# Autodesk Inventor assembly: Pata - Ensamble Trasero
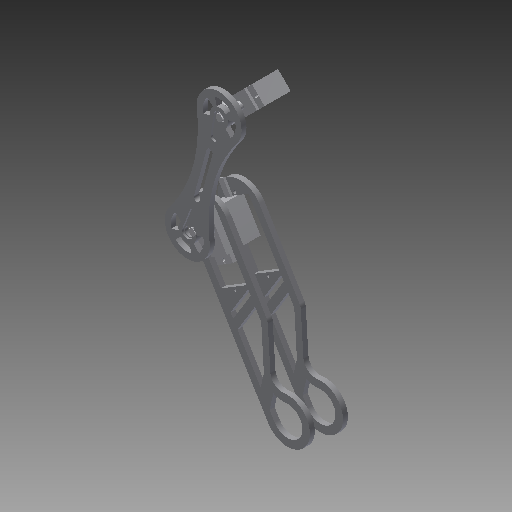
[picture p0: Inventor's stored thumbnail of the model, 512x512]
Saved by Autodesk Inventor 2019 (Build 230136000, 136)
## iProperties
Created: 2020-02-12
Part Number: Pata - Ensamble Trasero
Document SubType Name: Assembly
Designer: eddysanoli
Mass: 47.369 g
Surface Area: 327.582 cm^2
Volume: 47.369 cm^3
Density: 1 g/cm^3
Author: jacqu
## Documents named in this file (4)
- C:\Users\jacqu\Desktop\Robotica1_Proyecto-Cuadrupedo-master\Robotica1-Proyecto_Cuadrupedo\Pata - Ensamble Trasero.iam
- C:\Users\jacqu\Desktop\Robotica1_Proyecto-Cuadrupedo-master\Robotica1-Proyecto_Cuadrupedo\Pata - Brazo_MIR1_MIR.ipt
- C:\Users\jacqu\Desktop\Robotica1_Proyecto-Cuadrupedo-master\Robotica1-Proyecto_Cuadrupedo\Servo - Componente_MIR1_MIR.ipt
- C:\Users\jacqu\Desktop\Robotica1_Proyecto-Cuadrupedo-master\Robotica1-Proyecto_Cuadrupedo\Pata - Antebrazo.ipt
## Components (5 placed, 3 different names)
1. Pata - Antebrazo:1
2. Pata - Brazo_MIR1_MIR:1 — Coincidencia:1, Coincidencia:7, Coincidencia:8
3. Servo - Componente_MIR1_MIR:1 — Coincidencia:1, Coincidencia:7, Coincidencia:8, Coincidencia:9, Coincidencia:10, Nivelación:1
4. Servo - Componente_MIR1_MIR:2
5. Pata - Brazo_MIR1_MIR:2 — Coincidencia:9, Coincidencia:10, Nivelación:1
## Relationships (10: Mate 9, Flush 1)
- Coincidencia:1 [Mate]: Pata - Brazo_MIR1_MIR:1 ↔ Servo - Componente_MIR1_MIR:1
- Coincidencia:7 [Mate]: Pata - Brazo_MIR1_MIR:1 ↔ Servo - Componente_MIR1_MIR:1
- Coincidencia:8 [Mate]: Pata - Brazo_MIR1_MIR:1 ↔ Servo - Componente_MIR1_MIR:1
- [Mate]: Pata - Antebrazo:1 ↔ Servo - Componente_MIR1_MIR:1
- [Mate]: Pata - Antebrazo:1 ↔ Servo - Componente_MIR1_MIR:1
- [Mate]: Pata - Antebrazo:1 ↔ Servo - Componente_MIR1_MIR:2
- [Mate]: Pata - Antebrazo:1 ↔ Servo - Componente_MIR1_MIR:2
- Coincidencia:9 [Mate]: Servo - Componente_MIR1_MIR:1 ↔ Pata - Brazo_MIR1_MIR:2
- Coincidencia:10 [Mate]: Servo - Componente_MIR1_MIR:1 ↔ Pata - Brazo_MIR1_MIR:2
- Nivelación:1 [Flush]: Servo - Componente_MIR1_MIR:1 ↔ Pata - Brazo_MIR1_MIR:2
